# Autodesk Inventor assembly: Synchronous Belts Transmission
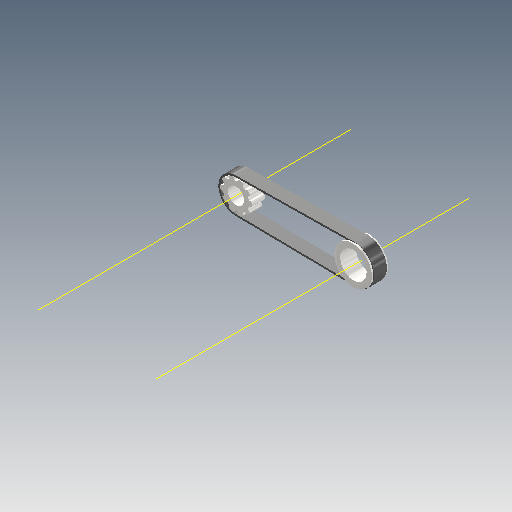
[picture p0: Inventor's stored thumbnail of the model, 512x512]
Saved by Autodesk Inventor 2020.3 (Build 243373010, 373A)
## iProperties
ClientObjectVersion: 1
Created: 2021-05-12
Part Number: Synchronous Belts Transmission
Document SubType Name: Assembly
Designer: marti
Author: marti
## Documents named in this file (4)
- C:\Users\marti\Documents\Inventor\RobotManipulateArm\17.4.2021 - Complete new IDEA\Head belt gear\Design Accelerator\Synchronous Belts Transmission3.iam
- C:\Users\marti\Documents\Inventor\RobotManipulateArm\17.4.2021 - Complete new IDEA\Head belt gear\Design Accelerator\Synchronous Belt3.ipt
- C:\Users\marti\Documents\Inventor\RobotManipulateArm\17.4.2021 - Complete new IDEA\Head belt gear\Design Accelerator\Synchronous Pulley13.ipt
- C:\Users\marti\Documents\Inventor\RobotManipulateArm\17.4.2021 - Complete new IDEA\Head belt gear\Design Accelerator\Synchronous Pulley23.ipt
## Components (3 placed, 3 different names)
1. Synchronous Belt:1 — Flush:1, Mate:1, Mate:2, Flush:2, Mate:3, Mate:4
2. Synchronous Pulley1:1 — Flush:1, Mate:1, Mate:2, Rotation:1
3. Synchronous Pulley2:1 — Flush:2, Mate:3, Rotation:1, Mate:4
## Relationships (7: Mate 4, Flush 2, RelateRotation 1)
- Flush:1: Synchronous Belt:1 ↔ Synchronous Pulley1:1
- Mate:1: Synchronous Belt:1 ↔ Synchronous Pulley1:1
- Mate:2: Synchronous Belt:1 ↔ Synchronous Pulley1:1
- Flush:2: Synchronous Belt:1 ↔ Synchronous Pulley2:1
- Mate:3: Synchronous Belt:1 ↔ Synchronous Pulley2:1
- Rotation:1 [RelateRotation] (1.1 ul): Synchronous Pulley1:1 ↔ Synchronous Pulley2:1
- Mate:4: Synchronous Belt:1 ↔ Synchronous Pulley2:1
